# Autodesk Inventor assembly: bowden extruder for printing
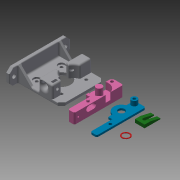
[picture p0: Inventor's stored thumbnail of the model, 180x180]
Saved by Autodesk Inventor 2014 (Build 180170000, 170)
## iProperties
Created: 2014-11-01
Part Number: bowden extruder for printing
Document SubType Name: Assembly
Designer: caleb
Author: caleb
## Documents named in this file (6)
- C:\cygwin\home\caleb\caleb-typea-settings\designs\bowden-extruder\bowden extruder for printing.iam
- C:\cygwin\home\caleb\caleb-typea-settings\designs\bowden-extruder\extruder base.ipt
- C:\cygwin\home\caleb\caleb-typea-settings\designs\bowden-extruder\tensioner 1.ipt
- C:\cygwin\home\caleb\caleb-typea-settings\designs\bowden-extruder\tensioner 2.ipt
- C:\cygwin\home\caleb\caleb-typea-settings\designs\bowden-extruder\tensioner washer.ipt
- C:\cygwin\home\caleb\caleb-typea-settings\designs\bowden-extruder\tension release wedge.ipt
## Components (5 placed, 5 different names)
1. extruder base:1 — Mate:1, Flush:1, Flush:2
2. tensioner 1:1 — Mate:2
3. tensioner 2:1 — Mate:3
4. tensioner washer:1 — Flush:1
5. tension release wedge:1 — Flush:2
## Relationships (5: Mate 3, Flush 2)
- Mate:1: extruder base:1
- Mate:2: tensioner 1:1
- Mate:3: tensioner 2:1
- Flush:1: extruder base:1 ↔ tensioner washer:1
- Flush:2: extruder base:1 ↔ tension release wedge:1
